# Autodesk Inventor assembly: LCD - AP203
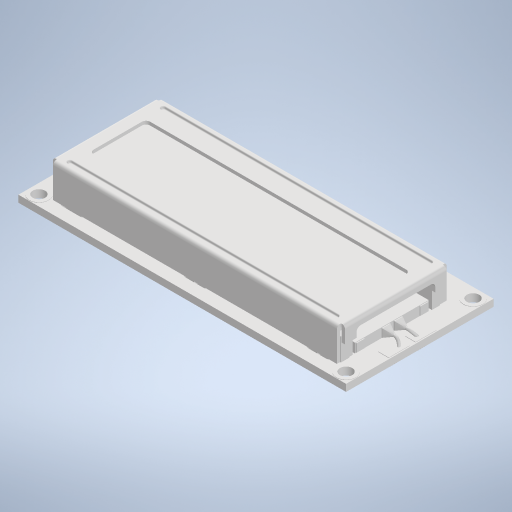
[picture p0: Inventor's stored thumbnail of the model, 512x512]
Saved by Autodesk Inventor 2024 (Build 280153000, 153)
## iProperties
Created: 2021-01-04
Part Number: LCD - AP203
Description: STEP AP203
Document SubType Name: Assembly
Designer: 5454s
Sending System: SolidWorks 2017
Preprocessor: SwSTEP 2.0
Title: LCD - AP203.STEP
Author: Arthur
Revision Number: ANY
## Documents named in this file (10)
- C:\Users\5454s\OneDrive\桌面\Smart_fan\LCD - AP203.iam
- C:\Users\5454s\OneDrive\桌面\16-x-2-lcd-display-module-with-iic-i2c-module-1.snapshot.2\LCD - AP203\pcbboard.ipt
- C:\Users\5454s\OneDrive\桌面\16-x-2-lcd-display-module-with-iic-i2c-module-1.snapshot.2\LCD - AP203\16pin_header__.ipt
- C:\Users\5454s\OneDrive\桌面\16-x-2-lcd-display-module-with-iic-i2c-module-1.snapshot.2\LCD - AP203\lcd window.ipt
- C:\Users\5454s\OneDrive\桌面\16-x-2-lcd-display-module-with-iic-i2c-module-1.snapshot.2\LCD - AP203\backlight.ipt
- C:\Users\5454s\OneDrive\桌面\16-x-2-lcd-display-module-with-iic-i2c-module-1.snapshot.2\LCD - AP203\conductor.ipt
- C:\Users\5454s\OneDrive\桌面\16-x-2-lcd-display-module-with-iic-i2c-module-1.snapshot.2\LCD - AP203\liquid crystal grabcad i2s.ipt
- C:\Users\5454s\OneDrive\桌面\16-x-2-lcd-display-module-with-iic-i2c-module-1.snapshot.2\LCD - AP203\smt_resistor222.ipt
- C:\Users\5454s\OneDrive\桌面\16-x-2-lcd-display-module-with-iic-i2c-module-1.snapshot.2\LCD - AP203\smt_resistor101.ipt
- C:\Users\5454s\OneDrive\桌面\16-x-2-lcd-display-module-with-iic-i2c-module-1.snapshot.2\LCD - AP203\i2c board.iam
## Components (16 placed, 16 different names)
1. pcbboard_1 — Mate:3, Mate:4
2. 16pin_header___2 — Mate:1, Mate:2, Mate:3, Mate:4
3. lcd window_3
4. backlight_4
5. conductor_5
6. conductor_6
7. liquid crystal grabcad i2s_7
8. smt_resistor222_8
9. smt_resistor222_9
10. smt_resistor222_10
11. smt_resistor222_11
12. smt_resistor222_12
13. smt_resistor222_13
14. smt_resistor101_14
15. smt_resistor101_15
16. i2c board_16 [sub-assembly] — Mate:1, Mate:2
## Relationships (4: Mate 4)
- Mate:1: 16pin_header___2 ↔ i2c board_16
- Mate:2: 16pin_header___2 ↔ i2c board_16
- Mate:3: pcbboard_1 ↔ 16pin_header___2
- Mate:4 (7 mm): pcbboard_1 ↔ 16pin_header___2
